# Autodesk Inventor assembly: Complete finger
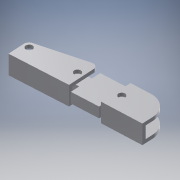
[picture p0: Inventor's stored thumbnail of the model, 180x180]
Saved by Autodesk Inventor 2018 (Build 220112000, 112)
## iProperties
Created: 2018-02-19
Part Number: Complete finger
Material: Générique
Document SubType Name: Assembly
Designer: Thomas
Author: Thomas
## Documents named in this file (4)
- D:\Users\Thomas\Desktop\Projet robot augmenté\robotConcept\Hand\Complete finger.iam
- D:\Users\Thomas\Desktop\Projet robot augmenté\robotConcept\Hand\Finger juncture.ipt
- D:\Users\Thomas\Desktop\Projet robot augmenté\robotConcept\Hand\finger1.ipt
- D:\Users\Thomas\Desktop\Projet robot augmenté\robotConcept\Hand\Finger2.ipt
## Components (3 placed, 3 different names)
1. Finger juncture:1 — Rotation:1, Rotation:2
2. finger1:1 — Rotation:1
3. Finger2:1 — Rotation:2
## Relationships (2: RevoluteJoint 2)
- Rotation:1 [RevoluteJoint]: Finger juncture:1 ↔ finger1:1
- Rotation:2 [RevoluteJoint]: Finger juncture:1 ↔ Finger2:1
